# Autodesk Inventor assembly: U assembly
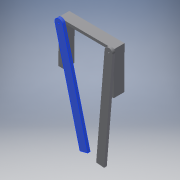
[picture p0: Inventor's stored thumbnail of the model, 180x180]
Saved by Autodesk Inventor 2019 (Build 230136000, 136)
## iProperties
Created: 2019-10-08
Part Number: U assembly
Document SubType Name: Assembly
Designer: Delta
Author: Delta
## Documents named in this file (3)
- C:\Robotics\2019-20_CAD\Collection\U assembly.iam
- C:\Robotics\2019-20_CAD\Collection\U-Part Gen 2.ipt
- C:\Robotics\2019-20_CAD\Collection\Wheel Arms.ipt
## Components (3 placed, 2 different names)
1. U-Part Gen 2:1 — Mate:1, Mate:2, Mate:3, Mate:4
2. Wheel Arms:1 — Mate:1, Mate:2
3. Wheel Arms:2 — Mate:3, Mate:4
## Relationships (4: Mate 4)
- Mate:1: U-Part Gen 2:1 ↔ Wheel Arms:1
- Mate:2: U-Part Gen 2:1 ↔ Wheel Arms:1
- Mate:3: U-Part Gen 2:1 ↔ Wheel Arms:2
- Mate:4: U-Part Gen 2:1 ↔ Wheel Arms:2
